# Autodesk Inventor assembly: Pillow Block with Bearing
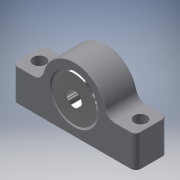
[picture p0: Inventor's stored thumbnail of the model, 180x180]
Saved by Autodesk Inventor 2016 (Build 200138000, 138)
## iProperties
Created: 2016-02-11
Part Number: Pillow Block with Bearing
Document SubType Name: Assembly
Designer: Spooner
Author: Spooner
## Documents named in this file (3)
- C:\Users\Spooner\Documents\Inventor\Bearing Pillow Block\Pillow Block with Bearing.iam
- C:\Users\Spooner\Documents\Inventor\Bearing Pillow Block\Bearing.ipt
- C:\Users\Spooner\Documents\Inventor\Bearing Pillow Block\Pillow Block.ipt
## Components (3 placed, 2 different names)
1. Bearing:1 — Flush:1, Flush:2, Insert:1
2. Pillow Block:1 — Flush:1, Flush:2
3. Bearing:2 — Insert:1
## Relationships (3: Flush 2, Insert 1)
- Flush:1: Bearing:1 ↔ Pillow Block:1
- Flush:2: Bearing:1 ↔ Pillow Block:1
- Insert:1: Bearing:1 ↔ Bearing:2
